# Autodesk Inventor assembly: Avionics
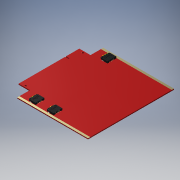
[picture p0: Inventor's stored thumbnail of the model, 180x180]
Saved by Autodesk Inventor 2018 (Build 220112000, 112)
## iProperties
Created: 2018-07-04
Part Number: Avionics
Document SubType Name: Assembly
Designer: Bradley
Mass: 9.58271 g
Surface Area: 172.214 cm^2
Volume: 8.40614 cm^3
Density: 1.13997 g/cm^3
Author: Bradley
## Documents named in this file (5)
- D:\Users\Bradley\Documents\CougsInSpace\CougSat1-Hardware\CougSat1-AvionicBoard\CADModel\Native\Avionics.iam
- D:\Users\Bradley\Documents\CougsInSpace\CougSat1-Hardware\CougSat1-AvionicBoard\CADModel\Native\Avionics_PCB.ipt
- D:\Users\Bradley\Documents\CougsInSpace\Resources\ComponentModels\Connectors\U.FL_Male.ipt
- D:\Users\Bradley\Documents\CougsInSpace\Resources\ComponentModels\Connectors\PicoLock-J-4.ipt
- D:\Users\Bradley\Documents\CougsInSpace\Resources\ComponentModels\Connectors\PicoLock-P-4.ipt
## Components (8 placed, 4 different names)
1. Avionics_PCB:1 — Mate:1, Mate:11, Mate:12, Mate:13
2. U.FL_Male:1 — Mate:1, Mate:2, Mate:3
3. PicoLock-J-4:1 — Mate:13, Flush:4, Flush:7, Mate:14
4. PicoLock-P-4:1
5. PicoLock-J-4:2 — Mate:11, Flush:5, Mate:15
6. PicoLock-P-4:2
7. PicoLock-J-4:3 — Mate:12, Flush:6, Flush:7
8. PicoLock-P-4:3
## Relationships (21: Mate 14, Flush 7)
- Mate:1: Avionics_PCB:1 ↔ U.FL_Male:1
- Mate:2 (85 mm): U.FL_Male:1
- Mate:3 (15 mm): U.FL_Male:1
- [Flush]: PicoLock-J-4:1 ↔ PicoLock-P-4:1
- [Mate]: PicoLock-J-4:1 ↔ PicoLock-P-4:1
- [Mate] (0.025 mm): PicoLock-J-4:1 ↔ PicoLock-P-4:1
- [Flush]: PicoLock-J-4:2 ↔ PicoLock-P-4:2
- [Mate]: PicoLock-J-4:2 ↔ PicoLock-P-4:2
- [Mate] (0.025 mm): PicoLock-J-4:2 ↔ PicoLock-P-4:2
- [Flush]: PicoLock-J-4:3 ↔ PicoLock-P-4:3
- [Mate]: PicoLock-J-4:3 ↔ PicoLock-P-4:3
- [Mate] (0.025 mm): PicoLock-J-4:3 ↔ PicoLock-P-4:3
- Mate:11: Avionics_PCB:1 ↔ PicoLock-J-4:2
- Mate:12: Avionics_PCB:1 ↔ PicoLock-J-4:3
- Mate:13: Avionics_PCB:1 ↔ PicoLock-J-4:1
- Flush:4 (-40 mm): PicoLock-J-4:1
- Flush:5 (40 mm): PicoLock-J-4:2
- Flush:6 (-40 mm): PicoLock-J-4:3
- Flush:7: PicoLock-J-4:1 ↔ PicoLock-J-4:3
- Mate:14 (30 mm): PicoLock-J-4:1
- Mate:15 (50 mm): PicoLock-J-4:2
## Named parameters: d6_d9 = 0 mm, d7_d10 = 0 mm, d8_d11 = 0.025 mm, d12_d9 = 0 mm, d13_d10 = 0 mm, d14_d11 = 0.025 mm
